# Autodesk Inventor assembly: Tail
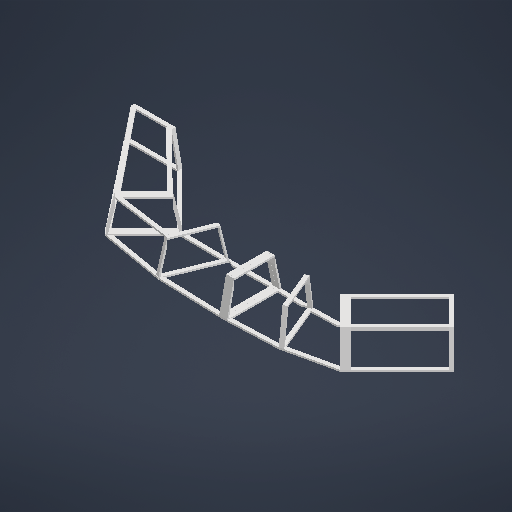
[picture p0: Inventor's stored thumbnail of the model, 512x512]
Saved by Autodesk Inventor 2026 (Build 300175000, 175)
## iProperties
Created: 2025-09-08
Part Number: Tail
Document SubType Name: Assembly
Designer: trott
Author: trott
## Documents named in this file (16)
- C:\Users\trott\Documents\UofSC-ASME-Tiger-Burn-Design-2025\CAD\Tail\Tail.iam
- C:\Users\trott\Documents\UofSC-ASME-Tiger-Burn-Design-2025\CAD\Tail\Struct_tail.iam
- C:\Users\trott\Documents\UofSC-ASME-Tiger-Burn-Design-2025\CAD\Tail\S_2x4x96.546.ipt
- C:\Users\trott\Documents\UofSC-ASME-Tiger-Burn-Design-2025\CAD\Tail\S_2x4x64.382.ipt
- C:\Users\trott\Documents\UofSC-ASME-Tiger-Burn-Design-2025\CAD\Tail\S_2x4x57.206.ipt
- C:\Users\trott\Documents\UofSC-ASME-Tiger-Burn-Design-2025\CAD\Tail\S_2x4x39.865.ipt
- C:\Users\trott\Documents\UofSC-ASME-Tiger-Burn-Design-2025\CAD\Tail\S_2x4x55.628.ipt
- C:\Users\trott\Documents\UofSC-ASME-Tiger-Burn-Design-2025\CAD\Tail\S_2x4x40.639.ipt
- C:\Users\trott\Documents\UofSC-ASME-Tiger-Burn-Design-2025\CAD\Tail\S_2x4x43.799.ipt
- C:\Users\trott\Documents\UofSC-ASME-Tiger-Burn-Design-2025\CAD\Tail\S_2x4x28.635.ipt
- C:\Users\trott\Documents\UofSC-ASME-Tiger-Burn-Design-2025\CAD\Tail\S_2x4x45.283.ipt
- C:\Users\trott\Documents\UofSC-ASME-Tiger-Burn-Design-2025\CAD\Tail\S_2x4x27.876.ipt
- C:\Users\trott\Documents\UofSC-ASME-Tiger-Burn-Design-2025\CAD\Tail\2x4x60.882.ipt
- C:\Users\trott\Documents\UofSC-ASME-Tiger-Burn-Design-2025\CAD\Tail\S_2x4x92.131.ipt
- C:\Users\trott\Documents\UofSC-ASME-Tiger-Burn-Design-2025\CAD\Tail\S_2x4x69.709.ipt
- C:\Users\trott\Documents\UofSC-ASME-Tiger-Burn-Design-2025\CAD\Tail\S_2x4x52.551.ipt
## Components (27 placed, 15 different names)
1. Struct_tail:1 [sub-assembly] — Mate:1, Mate:2, Flush:1, Mate:3, Mate:4, Flush:2, Mate:41, Mate:42, Flush:30, Mate:43, Flush:31, Mate:44
2. S_2x4x96.546:1 — Mate:1, Mate:2, Flush:1, Mate:6, Flush:3
3. S_2x4x64.382:1 — Mate:3, Mate:4, Flush:2, Mate:5
4. Struct_tail:2 [sub-assembly] — Mate:5, Mate:6, Flush:3, Mate:7, Flush:4, Flush:6, Mate:11
5. S_2x4x57.206:1 — Mate:8, Mate:9, Flush:5, Mate:13
6. Struct_tail:3 [sub-assembly] — Mate:7, Flush:4, Mate:8, Mate:9, Flush:5, Flush:6, Mate:10, Flush:7, Mate:45, Flush:32, Mate:46
7. S_2x4x39.865:1 — Mate:10, Flush:7, Mate:11, Mate:12, Flush:8
8. Struct_tail:4 [sub-assembly] — Mate:12, Flush:8, Mate:13, Mate:14, Flush:9, Mate:15, Mate:16, Mate:17, Flush:10
9. S_2x4x55.628:1 — Mate:14, Flush:9, Mate:15
10. S_2x4x40.639:1 — Mate:16, Mate:17, Flush:10, Mate:18, Flush:11, Mate:19
11. Struct_tail:5 [sub-assembly] — Mate:18, Flush:11, Mate:19, Mate:20, Flush:12, Flush:13
12. Struct_tail:6 [sub-assembly] — Mate:20, Flush:12, Flush:13, Mate:21, Mate:22, Flush:14, Mate:23, Mate:24, Flush:15
13. S_2x4x43.799:1 — Mate:21, Mate:22, Flush:14, Mate:25, Flush:16, Mate:26
14. S_2x4x28.635:1 — Mate:23, Mate:24, Flush:15
15. Struct_tail:7 [sub-assembly] — Mate:25, Flush:16, Mate:26, Mate:27, Mate:28, Flush:17, Mate:29, Mate:30, Flush:18
16. S_2x4x45.283:1 — Mate:27, Mate:28, Flush:17, Mate:31, Flush:19, Mate:32
17. S_2x4x27.876:1 — Mate:29, Mate:30, Flush:18
18. Struct_tail:8 [sub-assembly] — Mate:31, Flush:19, Mate:32, Mate:33, Flush:20, Flush:21
19. Struct_tail:9 [sub-assembly] — Mate:33, Flush:20, Flush:21, Mate:34, Flush:22, Flush:23, Mate:35, Flush:24, Flush:25, Mate:37, Flush:28, Mate:38, Mate:39, Flush:29, Mate:40
20. 2x4x60.882:1 — Mate:34, Flush:22, Flush:23, Mate:36, Flush:26, Flush:27
21. 2x4x60.882:2 — Mate:35, Flush:24, Flush:25
22. Struct_tail:10 [sub-assembly] — Mate:36, Flush:26, Flush:27
23. 2x4x60.882:3 — Mate:37, Flush:28, Mate:38
24. 2x4x60.882:4 — Mate:39, Flush:29, Mate:40
25. S_2x4x92.131:1 — Mate:41, Mate:42, Flush:30
26. S_2x4x69.709:1 — Mate:43, Flush:31, Mate:44
27. S_2x4x52.551:1 — Mate:45, Flush:32, Mate:46
## Relationships (78: Mate 46, Flush 32)
- Mate:1: Struct_tail:1 ↔ S_2x4x96.546:1
- Mate:2: Struct_tail:1 ↔ S_2x4x96.546:1
- Flush:1: Struct_tail:1 ↔ S_2x4x96.546:1
- Mate:3: Struct_tail:1 ↔ S_2x4x64.382:1
- Mate:4: Struct_tail:1 ↔ S_2x4x64.382:1
- Flush:2: Struct_tail:1 ↔ S_2x4x64.382:1
- Mate:5: S_2x4x64.382:1 ↔ Struct_tail:2
- Mate:6: S_2x4x96.546:1 ↔ Struct_tail:2
- Flush:3: S_2x4x96.546:1 ↔ Struct_tail:2
- Mate:7: Struct_tail:2 ↔ Struct_tail:3
- Flush:4: Struct_tail:2 ↔ Struct_tail:3
- Mate:8: S_2x4x57.206:1 ↔ Struct_tail:3
- Mate:9: S_2x4x57.206:1 ↔ Struct_tail:3
- Flush:5: S_2x4x57.206:1 ↔ Struct_tail:3
- Flush:6: Struct_tail:2 ↔ Struct_tail:3
- Mate:10: Struct_tail:3 ↔ S_2x4x39.865:1
- Flush:7: Struct_tail:3 ↔ S_2x4x39.865:1
- Mate:11: Struct_tail:2 ↔ S_2x4x39.865:1
- Mate:12: S_2x4x39.865:1 ↔ Struct_tail:4
- Flush:8: S_2x4x39.865:1 ↔ Struct_tail:4
- Mate:13: S_2x4x57.206:1 ↔ Struct_tail:4
- Mate:14: Struct_tail:4 ↔ S_2x4x55.628:1
- Flush:9: Struct_tail:4 ↔ S_2x4x55.628:1
- Mate:15: Struct_tail:4 ↔ S_2x4x55.628:1
- Mate:16: Struct_tail:4 ↔ S_2x4x40.639:1
- Mate:17: Struct_tail:4 ↔ S_2x4x40.639:1
- Flush:10: Struct_tail:4 ↔ S_2x4x40.639:1
- Mate:18: S_2x4x40.639:1 ↔ Struct_tail:5
- Flush:11: S_2x4x40.639:1 ↔ Struct_tail:5
- Mate:19: S_2x4x40.639:1 ↔ Struct_tail:5
- Mate:20: Struct_tail:5 ↔ Struct_tail:6
- Flush:12: Struct_tail:5 ↔ Struct_tail:6
- Flush:13: Struct_tail:5 ↔ Struct_tail:6
- Mate:21: Struct_tail:6 ↔ S_2x4x43.799:1
- Mate:22: Struct_tail:6 ↔ S_2x4x43.799:1
- Flush:14: Struct_tail:6 ↔ S_2x4x43.799:1
- Mate:23: Struct_tail:6 ↔ S_2x4x28.635:1
- Mate:24: Struct_tail:6 ↔ S_2x4x28.635:1
- Flush:15: Struct_tail:6 ↔ S_2x4x28.635:1
- Mate:25: S_2x4x43.799:1 ↔ Struct_tail:7
- Flush:16: S_2x4x43.799:1 ↔ Struct_tail:7
- Mate:26: S_2x4x43.799:1 ↔ Struct_tail:7
- Mate:27: Struct_tail:7 ↔ S_2x4x45.283:1
- Mate:28: Struct_tail:7 ↔ S_2x4x45.283:1
- Flush:17: Struct_tail:7 ↔ S_2x4x45.283:1
- Mate:29: Struct_tail:7 ↔ S_2x4x27.876:1
- Mate:30: Struct_tail:7 ↔ S_2x4x27.876:1
- Flush:18: Struct_tail:7 ↔ S_2x4x27.876:1
- Mate:31: S_2x4x45.283:1 ↔ Struct_tail:8
- Flush:19: S_2x4x45.283:1 ↔ Struct_tail:8
- Mate:32: S_2x4x45.283:1 ↔ Struct_tail:8
- Mate:33: Struct_tail:8 ↔ Struct_tail:9
- Flush:20: Struct_tail:8 ↔ Struct_tail:9
- Flush:21: Struct_tail:8 ↔ Struct_tail:9
- Mate:34: Struct_tail:9 ↔ 2x4x60.882:1
- Flush:22: Struct_tail:9 ↔ 2x4x60.882:1
- Flush:23: Struct_tail:9 ↔ 2x4x60.882:1
- Mate:35: Struct_tail:9 ↔ 2x4x60.882:2
- Flush:24: Struct_tail:9 ↔ 2x4x60.882:2
- Flush:25: Struct_tail:9 ↔ 2x4x60.882:2
- Mate:36: 2x4x60.882:1 ↔ Struct_tail:10
- Flush:26: 2x4x60.882:1 ↔ Struct_tail:10
- Flush:27: 2x4x60.882:1 ↔ Struct_tail:10
- Mate:37: Struct_tail:9 ↔ 2x4x60.882:3
- Flush:28: Struct_tail:9 ↔ 2x4x60.882:3
- Mate:38: Struct_tail:9 ↔ 2x4x60.882:3
- Mate:39: Struct_tail:9 ↔ 2x4x60.882:4
- Flush:29: Struct_tail:9 ↔ 2x4x60.882:4
- Mate:40: Struct_tail:9 ↔ 2x4x60.882:4
- Mate:41: Struct_tail:1 ↔ S_2x4x92.131:1
- Mate:42: Struct_tail:1 ↔ S_2x4x92.131:1
- Flush:30: Struct_tail:1 ↔ S_2x4x92.131:1
- Mate:43: Struct_tail:1 ↔ S_2x4x69.709:1
- Flush:31: Struct_tail:1 ↔ S_2x4x69.709:1
- Mate:44: Struct_tail:1 ↔ S_2x4x69.709:1
- Mate:45: Struct_tail:3 ↔ S_2x4x52.551:1
- Flush:32: Struct_tail:3 ↔ S_2x4x52.551:1
- Mate:46: Struct_tail:3 ↔ S_2x4x52.551:1
